# Autodesk Inventor assembly: 종아리발
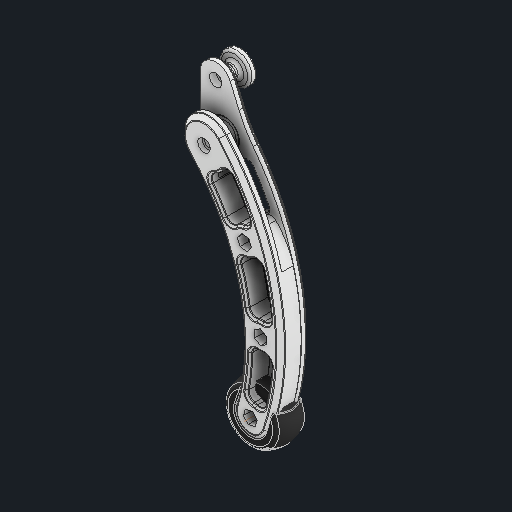
[picture p0: Inventor's stored thumbnail of the model, 512x512]
Saved by Autodesk Inventor 2027.1 (Build 311270010, 270A)
## iProperties
Created: 2026-08-22
Part Number: 종아리발
Document SubType Name: Assembly
Designer: moieboy9999
Mass: 19.8368 g
Surface Area: 219.095 cm^2
Volume: 30.8384 cm^3
Density: 0.643248 g/cm^3
Author: moieboy9999
## Documents named in this file (6)
- D:\micro_dog_cad\다리\프레임\왼종아리발.iam
- D:\micro_dog_cad\다리\프레임\발.ipt
- D:\micro_dog_cad\다리\프레임\종아리.ipt
- D:\micro_dog_cad\다리\프레임\링크축종아리.ipt
- D:\micro_dog_cad\다리\프레임\축종아리베어링고정.ipt
- D:\micro_dog_cad\다리\프레임\링크 고정.ipt
## Components (5 placed, 5 different names)
1. 발:1
2. 종아리:1
3. 링크축종아리:1
4. 축종아리베어링고정:1
5. 링크 고정:1
## Relationships (10: Mate 10)
- [Mate]: 링크축종아리:1 ↔ 축종아리베어링고정:1
- [Mate] (0.2 mm): 링크축종아리:1 ↔ 축종아리베어링고정:1
- [Mate]: 발:1 ↔ 종아리:1
- [Mate]: 발:1 ↔ 종아리:1
- [Mate]: 발:1 ↔ 종아리:1
- [Mate]: 종아리:1 ↔ 링크축종아리:1
- [Mate]: 종아리:1 ↔ 링크축종아리:1
- [Mate]: 종아리:1 ↔ 축종아리베어링고정:1
- [Mate]: 링크축종아리:1 ↔ 링크 고정:1
- [Mate]: 링크축종아리:1 ↔ 링크 고정:1
